# Autodesk Inventor assembly: body
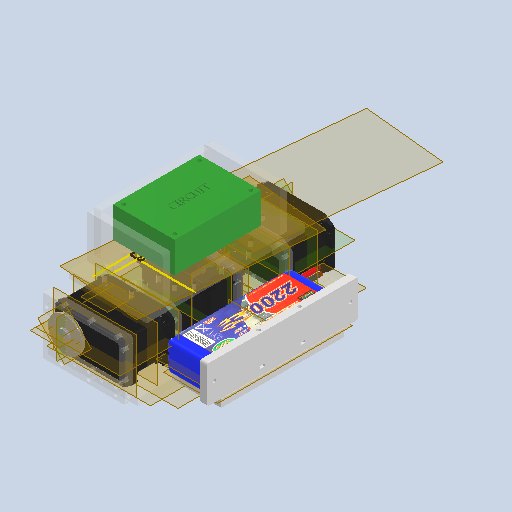
[picture p0: Inventor's stored thumbnail of the model, 512x512]
Saved by Autodesk Inventor 2024.3 (Build 283343000, 343)
## iProperties
Created: 2024-09-16
Part Number: body
Document SubType Name: Assembly
Designer: USER
Author: USER
## Documents named in this file (16)
- C:\Users\USER\Desktop\로빛 예비인턴\(git)19기 이원준 격투로봇 설계파일\upper_body\body.iam
- C:\Users\USER\Desktop\로빛 예비인턴\예비인턴 격투로봇 설계 프로젝트\격투로봇 백업 2\다이나믹셀\MX-64T.ipt
- C:\Users\USER\Desktop\로빛 예비인턴\예비인턴 격투로봇 설계 프로젝트\혼\64-106Horn.ipt
- C:\Users\USER\Desktop\로빛 예비인턴\예비인턴 격투로봇 설계 프로젝트\_idle-pelvis_adt.ipt
- C:\Users\USER\Desktop\로빛 예비인턴\(git)19기 이원준 격투로봇 설계파일\upper_body\_battery_adt_2_.ipt
- C:\Users\USER\Desktop\로빛 예비인턴\(git)19기 이원준 격투로봇 설계파일\upper_body\_battery_adt.ipt
- C:\Users\USER\Desktop\로빛 예비인턴\예비인턴 격투로봇 설계 프로젝트\Power_Control_inventor\Enrichpower_2200mAh_11.1V_30C.ipt
- C:\Users\USER\Desktop\로빛 예비인턴\(git)19기 이원준 격투로봇 설계파일\upper_body\_newbody1.ipt
- C:\Users\USER\Desktop\로빛 예비인턴\예비인턴 격투로봇 설계 프로젝트\격투로봇 백업 2\Motor_64_no_idle_ver.iam
- C:\Users\USER\Desktop\로빛 예비인턴\(git)19기 이원준 격투로봇 설계파일\upper_body\_face_froward_2.ipt
- C:\Users\USER\Desktop\로빛 예비인턴\(git)19기 이원준 격투로봇 설계파일\upper_body\_body_side_ver2.ipt
- C:\Users\USER\Desktop\로빛 예비인턴\(git)19기 이원준 격투로봇 설계파일\upper_body\_inner.ipt
- C:\Users\USER\Desktop\로빛 예비인턴\(git)19기 이원준 격투로봇 설계파일\upper_body\_body_3.ipt
- C:\Users\USER\Desktop\로빛 예비인턴\(git)19기 이원준 격투로봇 설계파일\upper_body\_head_adt_.ipt
- C:\Users\USER\Desktop\로빛 예비인턴\(git)19기 이원준 격투로봇 설계파일\upper_body\_head_adt_2.ipt
- C:\Users\USER\Desktop\로빛 예비인턴\(git)19기 이원준 격투로봇 설계파일\Power_Control_inventor\Circuit.ipt
## Components (19 placed, 15 different names)
1. _battery_adt_2_:1 — 각도:3
2. _idle-pelvis_adt:1
3. Enrichpower_2200mAh_11.1V_30C:1 — 각도:1, 메이트:1, 각도:3
4. _battery_adt:1 — 메이트:1
5. _newbody1:1 — 플러쉬:2, 플러쉬:3
6. _inner:1
7. _inner:2
8. _body_side_ver2:1 — 플러쉬:1
9. _body_side_ver2:2 — 플러쉬:3
10. _face_froward_2:1 — 각도:2
11. Motor_64_no_idle_ver:1 [sub-assembly]
12. Motor_64_no_idle_ver:2 [sub-assembly]
13. 64-106Horn:1
14. MX-64T:1
15. _body_3:1 — 삽입:1, 삽입:2, 삽입:3, 삽입:4, 삽입:5, 삽입:6, 삽입:7, 삽입:8
16. _head_adt_:1 — 삽입:1, 삽입:2, 삽입:3, 각도:2, 플러쉬:2
17. _head_adt_2:1 — 삽입:4, 삽입:5, 각도:1, 각도:4
18. _head_adt_2:2 — 삽입:6, 삽입:7, 플러쉬:1
19. Circuit:1 — 삽입:8, 각도:4
## Relationships (16: Insert 8, Angle 4, Flush 3, Mate 1)
- 삽입:1 [Insert]: _body_3:1 ↔ _head_adt_:1
- 삽입:2 [Insert]: _body_3:1 ↔ _head_adt_:1
- 삽입:3 [Insert]: _body_3:1 ↔ _head_adt_:1
- 삽입:4 [Insert]: _body_3:1 ↔ _head_adt_2:1
- 삽입:5 [Insert]: _body_3:1 ↔ _head_adt_2:1
- 삽입:6 [Insert]: _body_3:1 ↔ _head_adt_2:2
- 삽입:7 [Insert]: _body_3:1 ↔ _head_adt_2:2
- 각도:1 [Angle] (0 deg): Enrichpower_2200mAh_11.1V_30C:1 ↔ _head_adt_2:1
- 각도:2 [Angle] (0 deg): _face_froward_2:1 ↔ _head_adt_:1
- 플러쉬:1 [Flush] (37.375 mm): _body_side_ver2:1 ↔ _head_adt_2:2
- 플러쉬:2 [Flush]: _newbody1:1 ↔ _head_adt_:1
- 메이트:1 [Mate]: Enrichpower_2200mAh_11.1V_30C:1 ↔ _battery_adt:1
- 각도:3 [Angle] (0 deg): _battery_adt_2_:1 ↔ Enrichpower_2200mAh_11.1V_30C:1
- 삽입:8 [Insert] (10 mm): _body_3:1 ↔ Circuit:1
- 각도:4 [Angle] (0 deg): _head_adt_2:1 ↔ Circuit:1
- 플러쉬:3 [Flush]: _newbody1:1 ↔ _body_side_ver2:2
